# Autodesk Inventor assembly: Assembly1
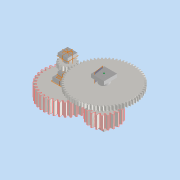
[picture p0: Inventor's stored thumbnail of the model, 180x180]
Saved by Autodesk Inventor 2022 (Build 260153000, 153)
## iProperties
Created: 2024-01-11
Part Number: Assembly1
Document SubType Name: Assembly
Designer: ktamu
Author: ktamu
## Documents named in this file (9)
- D:\SDinventor\SozoSekkeiEn1InventTryagainInvoForSubmit\Assembly1invo.iam
- D:\SDinventor\SozoSekkeiEn1InventTryagainInvoForSubmit\bearing1b.ipt
- D:\SDinventor\SozoSekkeiEn1InventTryagainInvoForSubmit\shaft1.ipt
- D:\SDinventor\SozoSekkeiEn1InventTryagainInvoForSubmit\bearing2b.ipt
- D:\SDinventor\SozoSekkeiEn1InventTryagainInvoForSubmit\shift2.ipt
- D:\SDinventor\SozoSekkeiEn1InventTryagainInvoForSubmit\bearing3b.ipt
- D:\SDinventor\SozoSekkeiEn1InventTryagainInvoForSubmit\shaft3.ipt
- D:\SDinventor\SozoSekkeiEn1InventTryagainInvoForSubmit\Assembly1invo\デザイン アクセラレータ\平歯車1.iam
- D:\SDinventor\SozoSekkeiEn1InventTryagainInvoForSubmit\Assembly1invo\デザイン アクセラレータ\平歯車auto1.iam
## Components (11 placed, 8 different names)
1. bearing1b:1 — フラッシュ:1, フラッシュ:2, フラッシュ:3, メイト:8
2. bearing1b:2 — フラッシュ:1, フラッシュ:2, フラッシュ:3, 回転:1, メイト:1, メイト:3, フラッシュ:5, メイト:4, メイト:9
3. shaft1:1 — 回転:1, 挿入:1, フラッシュ:13
4. bearing2b:1 — メイト:2, フラッシュ:5, メイト:4, メイト:5, メイト:6
5. bearing2b:2 — メイト:1, メイト:2, メイト:3, メイト:5, メイト:6, 角度:1, 回転:2, フラッシュ:11
6. shift2:1 — 角度:1, 回転:2, フラッシュ:14, 挿入:2, 挿入:3, フラッシュ:15, 挿入:4
7. bearing3b:1 — フラッシュ:11, メイト:8, メイト:9, フラッシュ:12, メイト:10, メイト:11, 回転:6
8. bearing3b:2 — フラッシュ:12, メイト:10, メイト:11
9. shaft3:1 — 回転:6, 挿入:5, フラッシュ:16
10. 平歯車auto:1 [sub-assembly] — 挿入:1, フラッシュ:13, フラッシュ:14, 挿入:2, 挿入:4
11. 平歯車autoB:1 [sub-assembly] — 挿入:3, フラッシュ:15, 挿入:5, フラッシュ:16
## Relationships (29: Flush 10, Mate 10, Insert 5, RevoluteJoint 3, Angle 1)
- フラッシュ:1 [Flush]: bearing1b:1 ↔ bearing1b:2
- フラッシュ:2 [Flush]: bearing1b:1 ↔ bearing1b:2
- フラッシュ:3 [Flush] (77 mm): bearing1b:1 ↔ bearing1b:2
- 回転:1 [RevoluteJoint]: bearing1b:2 ↔ shaft1:1
- メイト:1 [Mate]: bearing1b:2 ↔ bearing2b:2
- メイト:2 [Mate]: bearing2b:1 ↔ bearing2b:2
- メイト:3 [Mate]: bearing1b:2 ↔ bearing2b:2
- フラッシュ:5 [Flush]: bearing1b:2 ↔ bearing2b:1
- メイト:4 [Mate] (174 mm): bearing1b:2 ↔ bearing2b:1
- メイト:5 [Mate] (-210 mm): bearing2b:1 ↔ bearing2b:2
- メイト:6 [Mate]: bearing2b:1 ↔ bearing2b:2
- 角度:1 [Angle] (180 deg): bearing2b:2 ↔ shift2:1
- 回転:2 [RevoluteJoint]: bearing2b:2 ↔ shift2:1
- フラッシュ:11 [Flush]: bearing2b:2 ↔ bearing3b:1
- メイト:8 [Mate]: bearing1b:1 ↔ bearing3b:1
- メイト:9 [Mate] (-210 mm): bearing1b:2 ↔ bearing3b:1
- フラッシュ:12 [Flush]: bearing3b:1 ↔ bearing3b:2
- メイト:10 [Mate]: bearing3b:1 ↔ bearing3b:2
- メイト:11 [Mate] (-110 mm): bearing3b:1 ↔ bearing3b:2
- 回転:6 [RevoluteJoint]: bearing3b:1 ↔ shaft3:1
- 挿入:1 [Insert] (-32.5 mm): shaft1:1 ↔ 平歯車auto:1
- フラッシュ:13 [Flush]: shaft1:1 ↔ 平歯車auto:1
- フラッシュ:14 [Flush]: shift2:1 ↔ 平歯車auto:1
- 挿入:2 [Insert] (15 mm): shift2:1 ↔ 平歯車auto:1
- 挿入:3 [Insert] (5 mm): shift2:1 ↔ 平歯車autoB:1
- フラッシュ:15 [Flush]: shift2:1 ↔ 平歯車autoB:1
- 挿入:4 [Insert] (15 mm): shift2:1 ↔ 平歯車auto:1
- 挿入:5 [Insert] (5 mm): shaft3:1 ↔ 平歯車autoB:1
- フラッシュ:16 [Flush]: shaft3:1 ↔ 平歯車autoB:1
